# Autodesk Inventor assembly: lotka
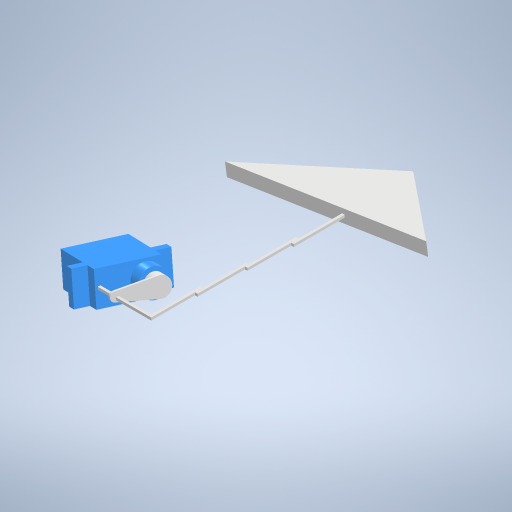
[picture p0: Inventor's stored thumbnail of the model, 512x512]
Saved by Autodesk Inventor 2023 (Build 270158000, 158)
## iProperties
Created: 2024-02-01
Part Number: lotka
Document SubType Name: Assembly
Designer: domin
Author: domin
## Documents named in this file (4)
- C:\Users\domin\Desktop\lotka.iam
- C:\Users\domin\Desktop\flap.ipt
- C:\Users\domin\Desktop\przewód.ipt
- C:\Users\domin\Desktop\serwo.ipt
## Components (7 placed, 3 different names)
1. flap:1 — Zestawiające:6
2. przewód:1 — Zestawiające:1, Zestawiające:2
3. serwo:1 — Zestawiające:1
4. przewód:4 — Zestawiające:5, Zestawiające:6
5. przewód:6 — Zestawiające:3, Zestawiające:4
6. przewód:7 — Zestawiające:4, Zestawiające:5
7. przewód:8 — Zestawiające:2, Zestawiające:3
## Relationships (6: Mate 6)
- Zestawiające:1 [Mate]: przewód:1 ↔ serwo:1
- Zestawiające:2 [Mate]: przewód:1 ↔ przewód:8
- Zestawiające:3 [Mate]: przewód:6 ↔ przewód:8
- Zestawiające:4 [Mate]: przewód:6 ↔ przewód:7
- Zestawiające:5 [Mate]: przewód:4 ↔ przewód:7
- Zestawiające:6 [Mate]: flap:1 ↔ przewód:4
